# Autodesk Inventor assembly: motor+tatakan
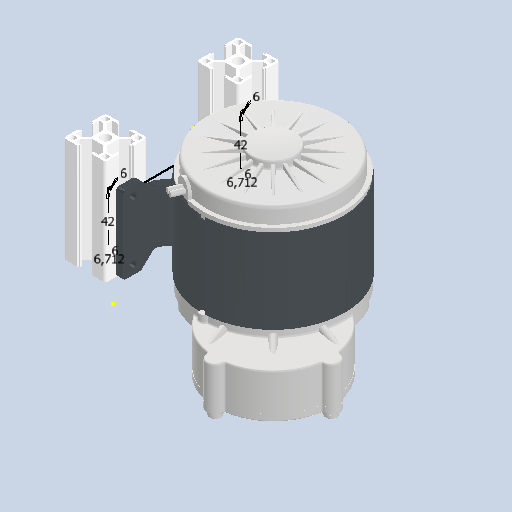
[picture p0: Inventor's stored thumbnail of the model, 512x512]
Saved by Autodesk Inventor 2023 (Build 270158000, 158)
## iProperties
Created: 2023-09-21
Part Number: motor+tatakan
Document SubType Name: Assembly
Designer: sigit
Author: sigit
## Documents named in this file (3)
- D:\Kuliah\SEMESTER 7\Robot Semprot\Design\2nd ROBOT\Assembly\motor+tatakan.iam
- D:\Kuliah\SEMESTER 7\Robot Semprot\Design\2nd ROBOT\Part\3030 75.ipt
- D:\Kuliah\SEMESTER 7\Robot Semprot\Design\2nd ROBOT\Assembly\Moteur DC - MY1016Z.iam
## Components (3 placed, 2 different names)
1. 3030 75:1 — Rotational:1
2. 3030 75:2 — Rotational:2
3. Moteur DC - MY1016Z:1 [sub-assembly] — Rotational:1, Rotational:2
## Relationships (2: RevoluteJoint 2)
- Rotational:1 [RevoluteJoint] (9.486 mm): 3030 75:1 ↔ Moteur DC - MY1016Z:1
- Rotational:2 [RevoluteJoint] (-9.486 mm): 3030 75:2 ↔ Moteur DC - MY1016Z:1
